# Autodesk Inventor assembly: Sneak100_Zeta
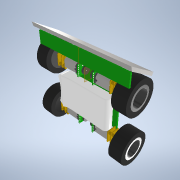
[picture p0: Inventor's stored thumbnail of the model, 180x180]
Saved by Autodesk Inventor 2021 (Build 250183000, 183)
## iProperties
Created: 2021-05-13
Part Number: Sneak100_Zeta
Document SubType Name: Assembly
Designer: ermoz
Author: ermoz
## Documents named in this file (7)
- D:\Moje Wyczyny\My_Poor_Projects\Sneak100_MiniSumo\minisumo-sneak100\mechanics\Sneak100_Zeta.iam
- D:\Moje Wyczyny\My_Poor_Projects\Sneak100_MiniSumo\minisumo-sneak100\mechanics\PreMadeParts\Pololu_MotorEncoderModule.iam
- D:\Moje Wyczyny\My_Poor_Projects\Sneak100_MiniSumo\minisumo-sneak100\mechanics\PreMadeParts\LiPO_2S_58x32x10.ipt
- D:\Moje Wyczyny\My_Poor_Projects\Sneak100_MiniSumo\minisumo-sneak100\mechanics\PreMadeParts\Solarbotics_RW2i.ipt
- D:\Moje Wyczyny\My_Poor_Projects\Sneak100_MiniSumo\minisumo-sneak100\mechanics\PreMadeParts\HM_Knife.ipt
- D:\Moje Wyczyny\My_Poor_Projects\Sneak100_MiniSumo\minisumo-sneak100\mechanics\ElectricElements\MainBoard.ipt
- D:\Moje Wyczyny\My_Poor_Projects\Sneak100_MiniSumo\minisumo-sneak100\mechanics\ElectricElements\SensorBoard.ipt
## Components (12 placed, 6 different names)
1. Pololu_MotorEncoderModule:1 [sub-assembly] — Mate:1, Flush:1, Flush:3, Flush:5, Angle:1, Mate:6, Mate:7, Symmetry:1
2. Pololu_MotorEncoderModule:2 [sub-assembly] — Mate:2, Flush:2, Flush:3, Flush:5, Angle:2, Mate:6, Mate:9, Mate:11, Mate:12, Mate:13
3. Pololu_MotorEncoderModule:3 [sub-assembly] — Mate:1, Flush:1, Flush:4, Mate:8, Symmetry:1
4. Pololu_MotorEncoderModule:4 [sub-assembly] — Mate:2, Flush:2, Flush:4, Mate:10, Mate:11
5. LiPO_2S_58x32x10:1
6. Solarbotics_RW2i:1 — Mate:3, Tangent:1, Flush:6, Mate:7, Flush:8, Symmetry:2
7. Solarbotics_RW2i:2 — Tangent:2, Mate:9, Flush:8
8. Solarbotics_RW2i:3 — Mate:3, Mate:8, Flush:7, Symmetry:2
9. Solarbotics_RW2i:4 — Mate:10, Flush:7
10. HM_Knife:1 — Mate:4, Flush:6, Mate:5, Angle:3
11. MainBoard:1 — Mate:12, Mate:13
12. SensorBoard:1 — Flush:9, Flush:10
## Relationships (31: Mate 14, Flush 10, Angle 3, Tangent 2, Symmetry 2)
- Mate:1: Pololu_MotorEncoderModule:1 ↔ Pololu_MotorEncoderModule:3
- Flush:1: Pololu_MotorEncoderModule:1 ↔ Pololu_MotorEncoderModule:3
- Mate:2: Pololu_MotorEncoderModule:2 ↔ Pololu_MotorEncoderModule:4
- Flush:2: Pololu_MotorEncoderModule:2 ↔ Pololu_MotorEncoderModule:4
- Flush:3: Pololu_MotorEncoderModule:1 ↔ Pololu_MotorEncoderModule:2
- Flush:4: Pololu_MotorEncoderModule:3 ↔ Pololu_MotorEncoderModule:4
- Flush:5: Pololu_MotorEncoderModule:1 ↔ Pololu_MotorEncoderModule:2
- Mate:3 (-98 mm): Solarbotics_RW2i:1 ↔ Solarbotics_RW2i:3
- Angle:1 (0 deg): Pololu_MotorEncoderModule:1
- Tangent:1: Solarbotics_RW2i:1
- Mate:4: HM_Knife:1
- Flush:6 (-1 mm): Solarbotics_RW2i:1 ↔ HM_Knife:1
- Angle:2 (0 deg): Pololu_MotorEncoderModule:2
- Tangent:2: Solarbotics_RW2i:2
- Mate:5 (-98 mm): HM_Knife:1
- Angle:3 (60 deg): HM_Knife:1
- Mate:6 (50 mm): Pololu_MotorEncoderModule:1 ↔ Pololu_MotorEncoderModule:2
- Mate:7: Pololu_MotorEncoderModule:1 ↔ Solarbotics_RW2i:1
- Mate:8: Pololu_MotorEncoderModule:3 ↔ Solarbotics_RW2i:3
- Mate:9: Pololu_MotorEncoderModule:2 ↔ Solarbotics_RW2i:2
- Mate:10: Pololu_MotorEncoderModule:4 ↔ Solarbotics_RW2i:4
- Flush:7: Solarbotics_RW2i:3 ↔ Solarbotics_RW2i:4
- Flush:8: Solarbotics_RW2i:1 ↔ Solarbotics_RW2i:2
- Mate:11 (-68 mm): Pololu_MotorEncoderModule:2 ↔ Pololu_MotorEncoderModule:4
- Symmetry:1: Pololu_MotorEncoderModule:1 ↔ Pololu_MotorEncoderModule:3
- Symmetry:2: Solarbotics_RW2i:1 ↔ Solarbotics_RW2i:3
- Mate:12 (2 mm): Pololu_MotorEncoderModule:2 ↔ MainBoard:1
- Mate:13: Pololu_MotorEncoderModule:2 ↔ MainBoard:1
- Flush:9 (4 mm): SensorBoard:1
- Flush:10 (-47 mm): SensorBoard:1
- Mate:14
